# Autodesk Inventor assembly: Solinoyd
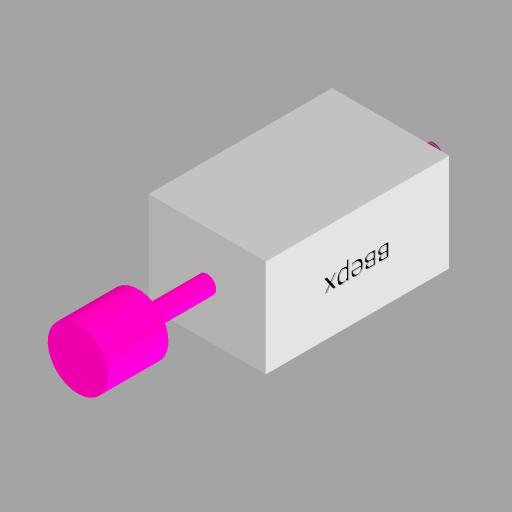
[picture p0: Inventor's stored thumbnail of the model, 512x512]
Saved by Autodesk Inventor 2024.2 (Build 282272000, 272)
## iProperties
Created: 2023-12-22
Part Number: Solinoyd
Document SubType Name: Assembly
Designer: Fedor Orlov
Author: Fedor Orlov
## Documents named in this file (3)
- C:\Users\Fedor Orlov\OneDrive\Robocup SSL\3D model\Solinoyd\Solinoyd.iam
- C:\Users\Fedor Orlov\OneDrive\Robocup SSL\3D model\Solinoyd\Solinoyd_telo.ipt
- C:\Users\Fedor Orlov\OneDrive\Robocup SSL\3D model\Solinoyd\Solinoyd_shtok.ipt
## Components (2 placed, 2 different names)
1. Solinoyd_telo:1 — Совмещение:1, Совмещение:2, Заподлицо:1, Совмещение:3, Совмещение:4
2. Solinoyd_shtok:1 — Совмещение:3, Совмещение:4
## Relationships (5: Mate 4, Flush 1)
- Совмещение:1 [Mate]: Solinoyd_telo:1
- Совмещение:2 [Mate]: Solinoyd_telo:1
- Заподлицо:1 [Flush]: Solinoyd_telo:1
- Совмещение:3 [Mate]: Solinoyd_telo:1 ↔ Solinoyd_shtok:1
- Совмещение:4 [Mate]: Solinoyd_telo:1 ↔ Solinoyd_shtok:1
